# Autodesk Inventor assembly: LowerBody_MIR
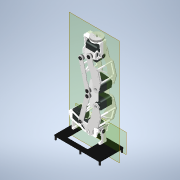
[picture p0: Inventor's stored thumbnail of the model, 180x180]
Saved by Autodesk Inventor 2020 (Build 240168000, 168)
## iProperties
Created: 2016-08-23
Part Number: LowerBody_MIR
Material: 一般
Document SubType Name: Assembly
Designer: Masato
Mass: 928.342 g
Surface Area: 2456.76 cm^2
Volume: 443.002 cm^3
Density: 2.09557 g/cm^3
Author: hiro
## Documents named in this file (12)
- C:\Users\Masato\Desktop\最新版\OpenPlatform_ver3_0\LowerBody_MIR.iam
- C:\Users\Masato\Desktop\最新版\OpenPlatform_ver3_0\下半身\付け根ロール\付け根ロール_1.iam
- C:\Users\Masato\Desktop\最新版\OpenPlatform_ver3_0\下半身\長穴減速\長穴減速_ホーン.iam
- C:\Users\Masato\Desktop\最新版\OpenPlatform_ver3_0\下半身\付け根\付け根_1.iam
- C:\Users\Masato\Desktop\最新版\OpenPlatform_ver3_0\下半身\リンク\UpperFrontLink.iam
- C:\Users\Masato\Desktop\最新版\OpenPlatform_ver3_0\下半身\リンク\UpperBackLink.iam
- C:\Users\Masato\Desktop\最新版\OpenPlatform_ver3_0\下半身\膝\膝_1.iam
- C:\Users\Masato\Desktop\最新版\OpenPlatform_ver3_0\下半身\リンク\LowerFrontLink.iam
- C:\Users\Masato\Desktop\最新版\OpenPlatform_ver3_0\下半身\リンク\LowerBackLink.iam
- C:\Users\Masato\Desktop\最新版\OpenPlatform_ver3_0\下半身\足首\足首_1.iam
- C:\Users\Masato\Desktop\最新版\OpenPlatform_ver3_0\下半身\足首\足首_独立ピッチ_1.iam
- C:\Users\Masato\Desktop\最新版\OpenPlatform_ver3_0\下半身\足裏\Foot_MIR.iam
## Components (12 placed, 11 different names)
1. 付け根ロール_1:1 [sub-assembly] — フラッシュ:26, フラッシュ:25, メイト:23, 挿入:97, 挿入:108, 挿入:107, 角度:4, 角度:12, 角度:4
2. 長穴減速_ホーン:1 [sub-assembly] — 挿入:97, 挿入:109
3. 付け根_1:1 [sub-assembly] — 挿入:109, 挿入:108, 挿入:107, 角度:4, 挿入:113, 挿入:112
4. UpperFrontLink:1 [sub-assembly] — 角度:12, 挿入:112, 挿入:111
5. UpperBackLink:1 [sub-assembly] — 挿入:114, 挿入:113
6. 膝_1:1 [sub-assembly] — 挿入:115, 挿入:98, 挿入:114, 挿入:111
7. LowerFrontLink:1 [sub-assembly] — 挿入:98, 挿入:118, 角度:3
8. LowerBackLink:1 [sub-assembly] — 挿入:115, 挿入:120, 挿入:122
9. 足首_1:1 [sub-assembly] — 挿入:119, 挿入:121, 挿入:16, 挿入:17
10. 足首_独立ピッチ_1:1 [sub-assembly] — 挿入:120, 挿入:119, 挿入:118
11. 足首_独立ピッチ_1:2 [sub-assembly] — 挿入:122, 挿入:121
12. Foot_MIR:1 [sub-assembly] — 挿入:16, 挿入:17, 角度:3, 角度:4
## Relationships (24: Insert 17, Angle 4, Mate 2, Flush 1)
- フラッシュ:26 [Flush]: 付け根ロール_1:1
- フラッシュ:25 [Mate]: 付け根ロール_1:1
- メイト:23 [Mate]: 付け根ロール_1:1
- 挿入:97 [Insert]: 付け根ロール_1:1 ↔ 長穴減速_ホーン:1
- 挿入:115 [Insert]: 膝_1:1 ↔ LowerBackLink:1
- 挿入:98 [Insert]: 膝_1:1 ↔ LowerFrontLink:1
- 挿入:109 [Insert]: 長穴減速_ホーン:1 ↔ 付け根_1:1
- 挿入:108 [Insert]: 付け根ロール_1:1 ↔ 付け根_1:1
- 挿入:107 [Insert]: 付け根ロール_1:1 ↔ 付け根_1:1
- 角度:4 [Angle] (0 deg): 付け根ロール_1:1 ↔ 付け根_1:1
- 挿入:114 [Insert]: UpperBackLink:1 ↔ 膝_1:1
- 挿入:113 [Insert]: 付け根_1:1 ↔ UpperBackLink:1
- 角度:12 [Angle] (-15 deg): 付け根ロール_1:1 ↔ UpperFrontLink:1
- 挿入:112 [Insert]: 付け根_1:1 ↔ UpperFrontLink:1
- 挿入:111 [Insert]: UpperFrontLink:1 ↔ 膝_1:1
- 挿入:120 [Insert]: LowerBackLink:1 ↔ 足首_独立ピッチ_1:1
- 挿入:119 [Insert]: 足首_1:1 ↔ 足首_独立ピッチ_1:1
- 挿入:118 [Insert]: LowerFrontLink:1 ↔ 足首_独立ピッチ_1:1
- 挿入:122 [Insert]: LowerBackLink:1 ↔ 足首_独立ピッチ_1:2
- 挿入:121 [Insert]: 足首_1:1 ↔ 足首_独立ピッチ_1:2
- 挿入:16 [Insert]: 足首_1:1 ↔ Foot_MIR:1
- 挿入:17 [Insert]: 足首_1:1 ↔ Foot_MIR:1
- 角度:3 [Angle] (15 deg): LowerFrontLink:1 ↔ Foot_MIR:1
- 角度:4 [Angle] (0 deg): 付け根ロール_1:1 ↔ Foot_MIR:1
